# Autodesk Inventor assembly: leg_under
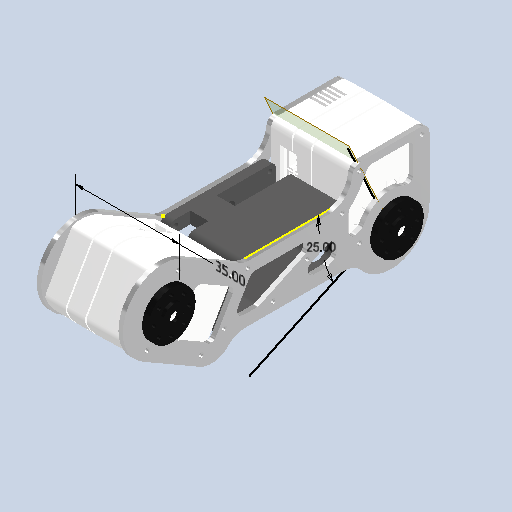
[picture p0: Inventor's stored thumbnail of the model, 512x512]
Saved by Autodesk Inventor 2024.1 (Build 281209000, 209)
## iProperties
Created: 2024-02-11
Part Number: leg_under
Document SubType Name: Assembly
Designer: hibik
Author: hibik
## Documents named in this file (5)
- C:\Users\hibik\Documents\Robomech\HR\Eglantyne\hard\leg\leg_under.iam
- C:\Users\hibik\Documents\Robomech\HR\Eglantyne\hard\leg\leg_under.ipt
- C:\Users\hibik\Desktop\ロボメカ\HR\2024.02.11 Rl\KRS3300モータ.ipt
- C:\Users\hibik\Desktop\ロボメカ\HR\2024.02.11 Rl\KRS3300サーボホーン.ipt
- C:\Users\hibik\Documents\Robomech\HR\Eglantyne\hard\leg\leg_under_middle.ipt
## Components (9 placed, 4 different names)
1. leg_under:1 — メイト:1, メイト:2, 角度:1, 挿入:9, 挿入:11, メイト:3, フラッシュ:1
2. leg_under:2 — 挿入:10, 挿入:12
3. KRS3300モータ:1 — 挿入:6, 挿入:8, メイト:1, 挿入:11, 挿入:12, メイト:4
4. KRS3300モータ:2 — 挿入:5, 挿入:7, メイト:2, 角度:1, 挿入:9, 挿入:10
5. KRS3300サーボホーン:1 — 挿入:5
6. KRS3300サーボホーン:2 — 挿入:6
7. KRS3300サーボホーン:3 — 挿入:8
8. KRS3300サーボホーン:4 — 挿入:7
9. leg_under_middle:1 — メイト:3, フラッシュ:1, メイト:4
## Relationships (14: Insert 8, Mate 4, Angle 1, Flush 1)
- 挿入:5 [Insert] (0.3 mm): KRS3300モータ:2 ↔ KRS3300サーボホーン:1
- 挿入:6 [Insert] (0.3 mm): KRS3300モータ:1 ↔ KRS3300サーボホーン:2
- 挿入:7 [Insert] (0.3 mm): KRS3300モータ:2 ↔ KRS3300サーボホーン:4
- 挿入:8 [Insert] (0.3 mm): KRS3300モータ:1 ↔ KRS3300サーボホーン:3
- メイト:1 [Mate]: leg_under:1 ↔ KRS3300モータ:1
- メイト:2 [Mate]: leg_under:1 ↔ KRS3300モータ:2
- 角度:1 [Angle] (0 deg): leg_under:1 ↔ KRS3300モータ:2
- 挿入:9 [Insert]: leg_under:1 ↔ KRS3300モータ:2
- 挿入:10 [Insert]: leg_under:2 ↔ KRS3300モータ:2
- 挿入:11 [Insert]: leg_under:1 ↔ KRS3300モータ:1
- 挿入:12 [Insert]: leg_under:2 ↔ KRS3300モータ:1
- メイト:3 [Mate]: leg_under:1 ↔ leg_under_middle:1
- フラッシュ:1 [Flush]: leg_under:1 ↔ leg_under_middle:1
- メイト:4 [Mate] (2 mm): KRS3300モータ:1 ↔ leg_under_middle:1
